# Autodesk Inventor assembly: Getriebe
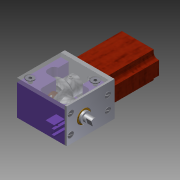
[picture p0: Inventor's stored thumbnail of the model, 180x180]
Saved by Autodesk Inventor 2014 SP1 (Build 180222100, 222)
## iProperties
Created: 2013-08-07
Part Number: Getriebe
Document SubType Name: Assembly
Designer: vogel
Author: vogel
## Documents named in this file (20)
- Z:\131087 - Tablet-Halterung\Getriebe.iam
- Z:\131087 - Tablet-Halterung\13_1087_010.ipt
- Z:\131087 - Tablet-Halterung\Kegelräder mädler 35550700.ipt
- Z:\131087 - Tablet-Halterung\Motor XDRIVE GM12F.ipt
- Z:\131087 - Tablet-Halterung\13_1087_012.ipt
- Z:\131087 - Tablet-Halterung\13_1087_013.ipt
- Z:\131087 - Tablet-Halterung\13_1087_014.ipt
- Z:\131087 - Tablet-Halterung\Sinterbuchse 364.ipt
- Z:\131087 - Tablet-Halterung\13_1087_021.ipt
- Z:\131087 - Tablet-Halterung\13_1087_027.ipt
- Z:\131087 - Tablet-Halterung\13_1087_015.ipt
- Z:\131087 - Tablet-Halterung\13_1087_022.ipt
- C:\Users\vogel.WWF-AD\Documents\Inventor\Content Center Files\R2014\de-DE\ISO 1207(2)\ISO 1207 - M1,6 x 6.ipt
- C:\Users\vogel.WWF-AD\Documents\Inventor\Content Center Files\R2014\de-DE\ISO 2009(2)\ISO 2009 - M2 x 6ISO 4.ipt
- C:\Users\vogel.WWF-AD\Documents\Inventor\Content Center Files\R2014\de-DE\ISO 2009(2)\ISO 2009 - M2 x 5ISO 3.ipt
- C:\Users\vogel.WWF-AD\Documents\Inventor\Content Center Files\R2014\de-DE\ISO 10642(1)\ISO 10642 - M3 x  8.ipt
- C:\Users\vogel.WWF-AD\Documents\Inventor\Content Center Files\R2014\de-DE\ISO 4766(1)\ISO 4766 - M2 x 2DIN EN.ipt
- C:\Users\vogel.WWF-AD\Documents\Inventor\Content Center Files\R2014\de-DE\ISO 4766(1)\ISO 4766 - M2 x 3DIN EN.ipt
- Z:\131087 - Tablet-Halterung\Sinterbuchse 35 60 325 61014.ipt
- C:\Users\vogel.WWF-AD\Documents\Inventor\Content Center Files\R2014\de-DE\ISO 4027\ISO 4027 - M3 x 4ISO.ipt
## Components (32 placed, 19 different names)
1. 13_1087_010:1 — Einfügen:3, Winkel:1, Passend:1, Fluchtend:2, Fluchtend:3, Passend:5, Fluchtend:4, Fluchtend:5, Einfügen:6, Passend:7, Fluchtend:6, Fluchtend:7, Einfügen:12
2. Kegelräder mädler 35550700:1 — Einfügen:3, Passend:30, Winkel:3, Passend:31
3. Kegelräder mädler 35550700:2 — Einfügen:5, Passend:28
4. Motor XDRIVE GM12F:1 — Winkel:1, Passend:2, Einfügen:5, Passend:4, Passend:6, Einfügen:7, Passend:25
5. Sinterbuchse 35 60 325 61014:1 — Einfügen:12, Einfügen:13
6. 13_1087_012:1 — Passend:1, Fluchtend:2, Passend:3, Fluchtend:3, Passend:4, Winkel:2, Passend:6, Einfügen:10, Einfügen:11, Passend:8, Passend:9, Passend:10, Passend:17, Passend:18, Passend:19, Passend:20
7. 13_1087_013:1 — Passend:2, Passend:3, Winkel:2
8. 13_1087_014:1 — Passend:5, Fluchtend:4, Fluchtend:5, Passend:15, Passend:16
9. Sinterbuchse 364:1 — Einfügen:6, Einfügen:9
10. 13_1087_021:1 — Passend:7, Fluchtend:6, Fluchtend:7, Passend:21, Passend:22, Passend:23, Passend:24
11. 13_1087_027:1 — Einfügen:7, Passend:26, Passend:29
12. 13_1087_015:1 — Einfügen:13, Winkel:3
13. 13_1087_022:1 — Einfügen:9, Passend:27, Fluchtend:8
14. ISO 1207 M1,6 x 6:1 — Einfügen:10
15. ISO 1207 M1,6 x 6:2 — Einfügen:11
16. ISO 2009 M2 x 6 x 4:1 — Passend:8
17. ISO 2009 M2 x 6 x 4:2 — Passend:9
18. ISO 2009 M2 x 6 x 4:3 — Passend:10
19. ISO 10642 M3 x  8:1 — Passend:15
20. ISO 10642 M3 x  8:2 — Passend:16
21. ISO 2009 M2 x 6 x 4:4 — Passend:17
22. ISO 2009 M2 x 6 x 4:5 — Passend:18
23. ISO 2009 M2 x 6 x 4:6 — Passend:19
24. ISO 2009 M2 x 6 x 4:7 — Passend:20
25. ISO 2009 M2 x 5 x 3:1 — Passend:21
26. ISO 2009 M2 x 5 x 3:2 — Passend:22
27. ISO 2009 M2 x 5 x 3:3 — Passend:23
28. ISO 2009 M2 x 5 x 3:4 — Passend:24
29. DIN EN 24766 M2 x 2:1 — Passend:25, Passend:26
30. DIN EN 24766 M2 x 3:1 — Passend:27, Fluchtend:8
31. ISO 4027 M3 x 4:1 — Passend:28, Passend:29
32. ISO 4027 M3 x 4:2 — Passend:30, Passend:31
## Relationships (46: Mate 27, Insert 9, Flush 7, Angle 3)
- Einfügen:3 [Insert] (1.6 mm): 13_1087_010:1 ↔ Kegelräder mädler 35550700:1
- Winkel:1 [Angle] (0 deg): 13_1087_010:1 ↔ Motor XDRIVE GM12F:1
- Passend:1 [Mate]: 13_1087_010:1 ↔ 13_1087_012:1
- Fluchtend:2 [Flush]: 13_1087_010:1 ↔ 13_1087_012:1
- Passend:2 [Mate]: Motor XDRIVE GM12F:1 ↔ 13_1087_013:1
- Einfügen:5 [Insert] (0.1 mm): Kegelräder mädler 35550700:2 ↔ Motor XDRIVE GM12F:1
- Passend:3 [Mate]: 13_1087_012:1 ↔ 13_1087_013:1
- Fluchtend:3 [Flush]: 13_1087_010:1 ↔ 13_1087_012:1
- Passend:4 [Mate]: Motor XDRIVE GM12F:1 ↔ 13_1087_012:1
- Winkel:2 [Angle] (0 deg): 13_1087_012:1 ↔ 13_1087_013:1
- Passend:5 [Mate]: 13_1087_010:1 ↔ 13_1087_014:1
- Fluchtend:4 [Flush]: 13_1087_010:1 ↔ 13_1087_014:1
- Fluchtend:5 [Flush]: 13_1087_010:1 ↔ 13_1087_014:1
- Passend:6 [Mate]: Motor XDRIVE GM12F:1 ↔ 13_1087_012:1
- Einfügen:6 [Insert]: 13_1087_010:1 ↔ Sinterbuchse 364:1
- Passend:7 [Mate]: 13_1087_010:1 ↔ 13_1087_021:1
- Fluchtend:6 [Flush]: 13_1087_010:1 ↔ 13_1087_021:1
- Fluchtend:7 [Flush]: 13_1087_010:1 ↔ 13_1087_021:1
- Einfügen:7 [Insert] (-3.5 mm): Motor XDRIVE GM12F:1 ↔ 13_1087_027:1
- Einfügen:9 [Insert]: Sinterbuchse 364:1 ↔ 13_1087_022:1
- Einfügen:10 [Insert]: 13_1087_012:1 ↔ ISO 1207 M1,6 x 6:1
- Einfügen:11 [Insert]: 13_1087_012:1 ↔ ISO 1207 M1,6 x 6:2
- Passend:8 [Mate]: 13_1087_012:1 ↔ ISO 2009 M2 x 6 x 4:1
- Passend:9 [Mate]: 13_1087_012:1 ↔ ISO 2009 M2 x 6 x 4:2
- Passend:10 [Mate]: 13_1087_012:1 ↔ ISO 2009 M2 x 6 x 4:3
- Passend:15 [Mate]: 13_1087_014:1 ↔ ISO 10642 M3 x  8:1
- Passend:16 [Mate]: 13_1087_014:1 ↔ ISO 10642 M3 x  8:2
- Passend:17 [Mate]: 13_1087_012:1 ↔ ISO 2009 M2 x 6 x 4:4
- Passend:18 [Mate]: 13_1087_012:1 ↔ ISO 2009 M2 x 6 x 4:5
- Passend:19 [Mate]: 13_1087_012:1 ↔ ISO 2009 M2 x 6 x 4:6
- Passend:20 [Mate]: 13_1087_012:1 ↔ ISO 2009 M2 x 6 x 4:7
- Passend:21 [Mate]: 13_1087_021:1 ↔ ISO 2009 M2 x 5 x 3:1
- Passend:22 [Mate]: 13_1087_021:1 ↔ ISO 2009 M2 x 5 x 3:2
- Passend:23 [Mate]: 13_1087_021:1 ↔ ISO 2009 M2 x 5 x 3:3
- Passend:24 [Mate]: 13_1087_021:1 ↔ ISO 2009 M2 x 5 x 3:4
- Passend:25 [Mate]: Motor XDRIVE GM12F:1 ↔ DIN EN 24766 M2 x 2:1
- Passend:26 [Mate]: 13_1087_027:1 ↔ DIN EN 24766 M2 x 2:1
- Passend:27 [Mate]: 13_1087_022:1 ↔ DIN EN 24766 M2 x 3:1
- Fluchtend:8 [Flush] (1 mm): 13_1087_022:1 ↔ DIN EN 24766 M2 x 3:1
- Einfügen:12 [Insert]: 13_1087_010:1 ↔ Sinterbuchse 35 60 325 61014:1
- Einfügen:13 [Insert]: Sinterbuchse 35 60 325 61014:1 ↔ 13_1087_015:1
- Passend:28 [Mate]: Kegelräder mädler 35550700:2 ↔ ISO 4027 M3 x 4:1
- Passend:29 [Mate] (2.5 mm): 13_1087_027:1 ↔ ISO 4027 M3 x 4:1
- Passend:30 [Mate]: Kegelräder mädler 35550700:1 ↔ ISO 4027 M3 x 4:2
- Winkel:3 [Angle] (0 deg): Kegelräder mädler 35550700:1 ↔ 13_1087_015:1
- Passend:31 [Mate] (2.5 mm): Kegelräder mädler 35550700:1 ↔ ISO 4027 M3 x 4:2
